# Autodesk Inventor assembly: F_Foot
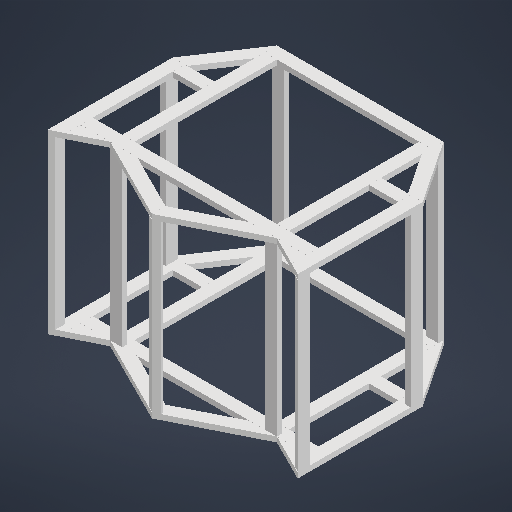
[picture p0: Inventor's stored thumbnail of the model, 512x512]
Saved by Autodesk Inventor 2026 (Build 300175000, 175)
## iProperties
Created: 2025-09-08
Part Number: F_Foot
Document SubType Name: Assembly
Designer: trott
Author: trott
## Documents named in this file (11)
- C:\Users\trott\Documents\UofSC-ASME-Tiger-Burn-Design-2025\CAD\Legs\Front Foot\F_Foot.iam
- C:\Users\trott\Documents\UofSC-ASME-Tiger-Burn-Design-2025\CAD\Legs\Front Foot\2x4x48.ipt
- C:\Users\trott\Documents\UofSC-ASME-Tiger-Burn-Design-2025\CAD\Legs\Front Foot\2x4x41.ipt
- C:\Users\trott\Documents\UofSC-ASME-Tiger-Burn-Design-2025\CAD\Legs\Front Foot\2x4x65.ipt
- C:\Users\trott\Documents\UofSC-ASME-Tiger-Burn-Design-2025\CAD\Legs\Front Foot\2x4x8.5.ipt
- C:\Users\trott\Documents\UofSC-ASME-Tiger-Burn-Design-2025\CAD\Legs\Front Foot\S_2x4x36.ipt
- C:\Users\trott\Documents\UofSC-ASME-Tiger-Burn-Design-2025\CAD\Legs\Front Foot\S_2x4x9.503.ipt
- C:\Users\trott\Documents\UofSC-ASME-Tiger-Burn-Design-2025\CAD\Legs\Front Foot\S_2x4x26.833.ipt
- C:\Users\trott\Documents\UofSC-ASME-Tiger-Burn-Design-2025\CAD\Legs\Front Foot\S2_2x4x48.ipt
- C:\Users\trott\Documents\UofSC-ASME-Tiger-Burn-Design-2025\CAD\Legs\Front Foot\S_2x4x48.ipt
- C:\Users\trott\Documents\UofSC-ASME-Tiger-Burn-Design-2025\CAD\Legs\Front Foot\S_2x4x21.633.ipt
## Components (37 placed, 10 different names)
1. 2x4x48:7 — Mate:17, Flush:23, Flush:24
2. 2x4x48:8 — Mate:18, Flush:25, Flush:26
3. S2_2x4x48:1 — Mate:19, Flush:27, Flush:28
4. S_2x4x48:1 — Mate:20, Flush:29, Flush:30
5. S_2x4x48:2 — Mate:21, Flush:31, Flush:32
6. 2x4x48:2 — Mate:16, Flush:21, Flush:22
7. 2x4x48:3
8. 2x4x48:4
9. 2x4x48:5
10. 2x4x65:1 — Mate:3, Flush:5, Flush:6, Flush:7, Mate:6, Flush:13, Mate:7, Flush:15, Mate:9, Mate:11, Mate:12, Flush:19, Mate:15, Flush:20
11. S_2x4x9.503:2 — Mate:10, Mate:11, Flush:18
12. S_2x4x36:2 — Mate:7, Flush:15, Flush:16, Mate:10, Flush:18, Mate:18, Flush:25, Flush:26
13. 2x4x8.5:2 — Mate:5, Flush:11, Flush:12, Flush:16
14. 2x4x41:2 — Mate:2, Flush:3, Flush:4, Mate:3, Flush:5, Mate:5, Flush:11
15. S_2x4x26.833:2 — Mate:14, Mate:15, Flush:20, Flush:27
16. S_2x4x26.833:1 — Mate:12, Mate:13, Flush:19, Mate:14, Mate:19, Flush:28
17. S_2x4x36:1 — Mate:6, Flush:13, Flush:14, Mate:8, Flush:17, Mate:17, Flush:23, Flush:24
18. S_2x4x9.503:1 — Mate:8, Flush:17, Mate:9, Mate:13
19. 2x4x41:1 — Mate:1, Flush:1, Flush:2, Flush:6, Flush:7, Mate:4, Flush:8, Flush:10
20. 2x4x8.5:1 — Mate:4, Flush:8, Flush:9, Flush:10, Flush:14
21. 2x4x48:1 — Mate:1, Flush:1, Flush:2, Mate:2, Flush:3, Flush:4, Flush:9, Flush:12, Mate:16, Flush:21, Flush:22
22. 2x4x65:2
23. S_2x4x9.503:3
24. S_2x4x36:3 — Mate:21, Flush:31, Flush:32, Mate:25
25. 2x4x8.5:3
26. 2x4x41:3 — Flush:34
27. S_2x4x26.833:3
28. S_2x4x26.833:4
29. S_2x4x36:4 — Mate:20, Flush:29, Flush:30, Mate:22, Flush:33
30. S_2x4x9.503:4
31. 2x4x41:4
32. 2x4x8.5:4
33. 2x4x48:6 — Mate:23, Mate:24
34. S_2x4x21.633:1 — Mate:22, Flush:33, Mate:23
35. S_2x4x21.633:2 — Mate:24, Mate:25, Flush:34
36. S_2x4x21.633:3
37. S_2x4x21.633:4
## Component patterns: (4 elements, first: 2x4x48:2), (2 elements, first: 2x4x65:1 + S_2x4x9.503:2 + S_2x4x36:2 + 2x4x8.5:2 + 2x4x41:2 + S_2x4x26.833:2 + S_2x4x26.833:1 + S_2x4x36:1 + S_2x4x9.503:1 + 2x4x41:1 + 2x4x8.5:1 + 2x4x48:1), (2 elements, first: S_2x4x21.633:1 + S_2x4x21.633:2)
## Relationships (59: Flush 34, Mate 25)
- Mate:1: 2x4x41:1 ↔ 2x4x48:1
- Flush:1: 2x4x41:1 ↔ 2x4x48:1
- Flush:2: 2x4x41:1 ↔ 2x4x48:1
- Mate:2: 2x4x41:2 ↔ 2x4x48:1
- Flush:3: 2x4x41:2 ↔ 2x4x48:1
- Flush:4: 2x4x41:2 ↔ 2x4x48:1
- Mate:3: 2x4x65:1 ↔ 2x4x41:2
- Flush:5: 2x4x65:1 ↔ 2x4x41:2
- Flush:6: 2x4x65:1 ↔ 2x4x41:1
- Flush:7 (-215.9 mm): 2x4x65:1 ↔ 2x4x41:1
- Mate:4: 2x4x41:1 ↔ 2x4x8.5:1
- Flush:8: 2x4x41:1 ↔ 2x4x8.5:1
- Flush:9 (457.2 mm): 2x4x8.5:1 ↔ 2x4x48:1
- Flush:10: 2x4x41:1 ↔ 2x4x8.5:1
- Mate:5: 2x4x8.5:2 ↔ 2x4x41:2
- Flush:11: 2x4x8.5:2 ↔ 2x4x41:2
- Flush:12 (457.2 mm): 2x4x8.5:2 ↔ 2x4x48:1
- Mate:6: 2x4x65:1 ↔ S_2x4x36:1
- Flush:13: 2x4x65:1 ↔ S_2x4x36:1
- Flush:14: S_2x4x36:1 ↔ 2x4x8.5:1
- Mate:7: 2x4x65:1 ↔ S_2x4x36:2
- Flush:15: 2x4x65:1 ↔ S_2x4x36:2
- Flush:16: S_2x4x36:2 ↔ 2x4x8.5:2
- Mate:8: S_2x4x36:1 ↔ S_2x4x9.503:1
- Flush:17: S_2x4x36:1 ↔ S_2x4x9.503:1
- Mate:9: 2x4x65:1 ↔ S_2x4x9.503:1
- Mate:10: S_2x4x9.503:2 ↔ S_2x4x36:2
- Mate:11: 2x4x65:1 ↔ S_2x4x9.503:2
- Flush:18: S_2x4x9.503:2 ↔ S_2x4x36:2
- Mate:12: 2x4x65:1 ↔ S_2x4x26.833:1
- Mate:13: S_2x4x26.833:1 ↔ S_2x4x9.503:1
- Flush:19: 2x4x65:1 ↔ S_2x4x26.833:1
- Mate:14: S_2x4x26.833:2 ↔ S_2x4x26.833:1
- Mate:15: 2x4x65:1 ↔ S_2x4x26.833:2
- Flush:20: 2x4x65:1 ↔ S_2x4x26.833:2
- Mate:16: 2x4x48:2 ↔ 2x4x48:1
- Flush:21: 2x4x48:2 ↔ 2x4x48:1
- Flush:22: 2x4x48:2 ↔ 2x4x48:1
- Mate:17: 2x4x48:7 ↔ S_2x4x36:1
- Flush:23: 2x4x48:7 ↔ S_2x4x36:1
- Flush:24: 2x4x48:7 ↔ S_2x4x36:1
- Mate:18: 2x4x48:8 ↔ S_2x4x36:2
- Flush:25: 2x4x48:8 ↔ S_2x4x36:2
- Flush:26: 2x4x48:8 ↔ S_2x4x36:2
- Mate:19: S2_2x4x48:1 ↔ S_2x4x26.833:1
- Flush:27: S2_2x4x48:1 ↔ S_2x4x26.833:2
- Flush:28: S2_2x4x48:1 ↔ S_2x4x26.833:1
- Mate:20: S_2x4x48:1 ↔ S_2x4x36:4
- Flush:29: S_2x4x48:1 ↔ S_2x4x36:4
- Flush:30: S_2x4x48:1 ↔ S_2x4x36:4
- Mate:21: S_2x4x48:2 ↔ S_2x4x36:3
- Flush:31: S_2x4x48:2 ↔ S_2x4x36:3
- Flush:32: S_2x4x48:2 ↔ S_2x4x36:3
- Mate:22: S_2x4x36:4 ↔ S_2x4x21.633:1
- Flush:33: S_2x4x36:4 ↔ S_2x4x21.633:1
- Mate:23: 2x4x48:6 ↔ S_2x4x21.633:1
- Mate:24: 2x4x48:6 ↔ S_2x4x21.633:2
- Mate:25: S_2x4x36:3 ↔ S_2x4x21.633:2
- Flush:34: 2x4x41:3 ↔ S_2x4x21.633:2
